# Autodesk Inventor assembly: Bottom Assembly
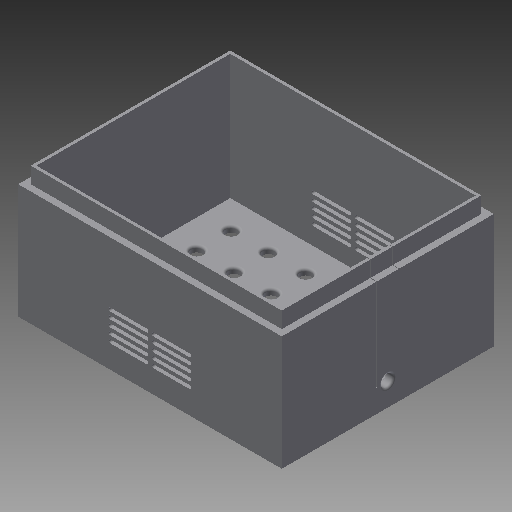
[picture p0: Inventor's stored thumbnail of the model, 512x512]
Saved by Autodesk Inventor 2017 (Build 210142000, 142)
## iProperties
Created: 2018-03-22
Part Number: Bottom Assembly
Document SubType Name: Assembly
Designer: Arjuna
Author: Arjuna
## Documents named in this file (3)
- D:\Users\Arjuna\Documents\NTU\FYP\Hardware\Bottom Assembly.iam
- D:\Users\Arjuna\Documents\NTU\FYP\Hardware\Bottom.ipt
- D:\Users\Arjuna\Documents\NTU\FYP\Hardware\Bottom Clip.ipt
## Components (2 placed, 2 different names)
1. Bottom:1 — Flush:1, Flush:2, Flush:3, Flush:4, Flush:6
2. BOttom Clip:1 — Flush:4, Flush:5, Flush:6
## Relationships (6: Flush 6)
- Flush:1: Bottom:1
- Flush:2: Bottom:1
- Flush:3: Bottom:1
- Flush:4: Bottom:1 ↔ BOttom Clip:1
- Flush:5: BOttom Clip:1
- Flush:6: Bottom:1 ↔ BOttom Clip:1
